# Autodesk Inventor assembly: CollectorPrototype
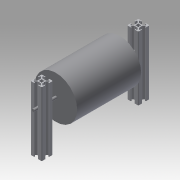
[picture p0: Inventor's stored thumbnail of the model, 180x180]
Saved by Autodesk Inventor 2016 (Build 200138000, 138)
## iProperties
Created: 2016-12-07
Part Number: CollectorPrototype
Document SubType Name: Assembly
Designer: Delta
Author: Delta
## Documents named in this file (5)
- C:\Robotics\CAD\2016-17_CAD\CollectorPrototype.iam
- C:\Robotics\CAD\COTSParts\Bosch Extrusion\Bosch 20x20 - 4.5 Part.Shoot.ipt
- C:\Robotics\CAD\2016-17_CAD\6InchAx.ipt
- C:\Robotics\CAD\2016-17_CAD\CollectorBrush.ipt
- C:\Robotics\CAD\COTSParts\Actobotics\615 parts\615102.ipt
## Components (5 placed, 4 different names)
1. Bosch 20x20 - 4.5 Part.Shoot:2 — Insert:1
2. 6InchAx:1 — Insert:1, Insert:2, Insert:3, Mate:2
3. CollectorBrush:1 — Insert:3, Mate:1
4. 615102:1 — Mate:1, Mate:2
5. Bosch 20x20 - 4.5 Part.Shoot:3 — Insert:2
## Relationships (5: Insert 3, Mate 2)
- Insert:1 (-10.8966 mm): Bosch 20x20 - 4.5 Part.Shoot:2 ↔ 6InchAx:1
- Insert:2 (10.8966 mm): 6InchAx:1 ↔ Bosch 20x20 - 4.5 Part.Shoot:3
- Insert:3 (40.64 mm): 6InchAx:1 ↔ CollectorBrush:1
- Mate:1: CollectorBrush:1 ↔ 615102:1
- Mate:2: 6InchAx:1 ↔ 615102:1
